# Autodesk Inventor assembly: ПД Модуль 200х140х75
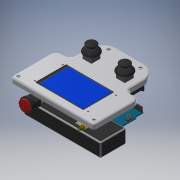
[picture p0: Inventor's stored thumbnail of the model, 180x180]
Saved by Autodesk Inventor 2019 (Build 230136000, 136)
## iProperties
Created: 2020-05-19
Part Number: ПД Модуль 200х140х75
Material: Типовые
Document SubType Name: Assembly
Designer: Surflay
Author: Surflay
## Documents named in this file (9)
- C:\Users\bossl\Desktop\Модуль ДУ Inventor\Дистанционная связь (модуль)\ПД Сборка ДУ 150х140х65.iam
- C:\Users\bossl\Desktop\Модуль ДУ Inventor\Дистанционная связь (модуль)\ПД Коробка 150х140х65.ipt
- C:\Users\bossl\Desktop\Модуль ДУ Inventor\Дистанционная связь (модуль)\РадиоМодуль.ipt
- C:\Users\bossl\Desktop\Модуль ДУ Inventor\Дистанционная связь (модуль)\Arduino UNO.ipt
- C:\Users\bossl\Desktop\Модуль ДУ Inventor\Дистанционная связь (модуль)\Аккумулятор.ipt
- C:\Users\bossl\Desktop\Модуль ДУ Inventor\Дистанционная связь (модуль)\Кнопка.ipt
- C:\Users\bossl\Desktop\Модуль ДУ Inventor\Дистанционная связь (модуль)\ВольтметрЦифровой.ipt
- C:\Users\bossl\Desktop\Модуль ДУ Inventor\Дистанционная связь (модуль)\NextionDisplay.ipt
- C:\Users\bossl\Desktop\Модуль ДУ Inventor\Дистанционная связь (модуль)\Джойстик.ipt
## Components (9 placed, 8 different names)
1. ПД Коробка 150х140х65:1 — Совмещение:1, Совмещение:2, Совмещение:3, Совмещение:4, Совмещение:6, Совмещение:9, Совмещение:10, Совмещение:11, Совмещение:12, Совмещение:13, Совмещение:15, Совмещение:16, Совмещение:17, Совмещение:18, Совмещение:19, Совмещение:20, Совмещение:21, Совмещение:23, Совмещение:24, Совмещение:25
2. РадиоМодуль:1 — Совмещение:23, Совмещение:24, Совмещение:25
3. Arduino UNO:1 — Совмещение:11, Совмещение:12, Совмещение:13
4. Аккумулятор:1 — Совмещение:4, Совмещение:9, Совмещение:10
5. Кнопка:1 — Совмещение:6, Совмещение:15, Совмещение:16
6. ВольтметрЦифровой:1 — Совмещение:1, Совмещение:2, Совмещение:3
7. NextionDisplay:1 — Совмещение:17, Совмещение:18, Совмещение:19, Совмещение:22
8. Джойстик:1
9. Джойстик:2 — Совмещение:20, Совмещение:21, Совмещение:22
## Component patterns: (2 elements, first: Джойстик:1)
## Relationships (21: Mate 21)
- Совмещение:1 [Mate]: ПД Коробка 150х140х65:1 ↔ ВольтметрЦифровой:1
- Совмещение:2 [Mate] (18.75 mm): ПД Коробка 150х140х65:1 ↔ ВольтметрЦифровой:1
- Совмещение:3 [Mate] (0.604 mm): ПД Коробка 150х140х65:1 ↔ ВольтметрЦифровой:1
- Совмещение:4 [Mate]: ПД Коробка 150х140х65:1 ↔ Аккумулятор:1
- Совмещение:6 [Mate]: ПД Коробка 150х140х65:1 ↔ Кнопка:1
- Совмещение:9 [Mate] (12 mm): ПД Коробка 150х140х65:1 ↔ Аккумулятор:1
- Совмещение:10 [Mate]: ПД Коробка 150х140х65:1 ↔ Аккумулятор:1
- Совмещение:11 [Mate] (5 mm): ПД Коробка 150х140х65:1 ↔ Arduino UNO:1
- Совмещение:12 [Mate] (25 mm): ПД Коробка 150х140х65:1 ↔ Arduino UNO:1
- Совмещение:13 [Mate] (17 mm): ПД Коробка 150х140х65:1 ↔ Arduino UNO:1
- Совмещение:15 [Mate] (20 mm): ПД Коробка 150х140х65:1 ↔ Кнопка:1
- Совмещение:16 [Mate] (30 mm): ПД Коробка 150х140х65:1 ↔ Кнопка:1
- Совмещение:17 [Mate]: ПД Коробка 150х140х65:1 ↔ NextionDisplay:1
- Совмещение:18 [Mate] (29.25 mm): ПД Коробка 150х140х65:1 ↔ NextionDisplay:1
- Совмещение:19 [Mate] (10 mm): ПД Коробка 150х140х65:1 ↔ NextionDisplay:1
- Совмещение:20 [Mate]: ПД Коробка 150х140х65:1 ↔ Джойстик:2
- Совмещение:21 [Mate] (29.5 mm): ПД Коробка 150х140х65:1 ↔ Джойстик:2
- Совмещение:22 [Mate] (20 mm): NextionDisplay:1 ↔ Джойстик:2
- Совмещение:23 [Mate] (10 mm): ПД Коробка 150х140х65:1 ↔ РадиоМодуль:1
- Совмещение:24 [Mate]: ПД Коробка 150х140х65:1 ↔ РадиоМодуль:1
- Совмещение:25 [Mate] (15 mm): ПД Коробка 150х140х65:1 ↔ РадиоМодуль:1
